# Autodesk Inventor assembly: UltrasonicAssembly
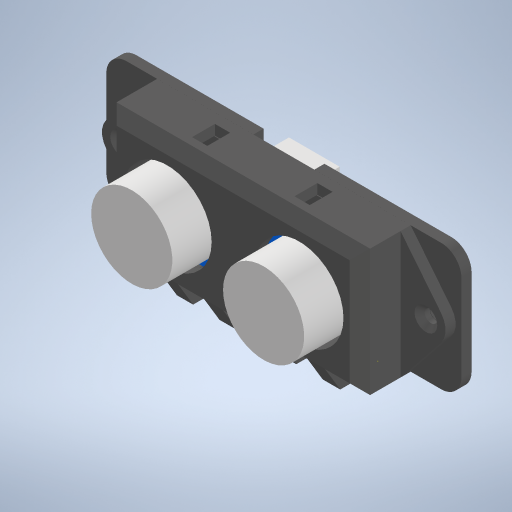
[picture p0: Inventor's stored thumbnail of the model, 512x512]
Saved by Autodesk Inventor 2024.2 (Build 282272000, 272)
## iProperties
Created: 2024-05-04
Part Number: UltrasonicAssembly
Document SubType Name: Assembly
Designer: ringl
Author: ringl
## Documents named in this file (4)
- C:\Users\ringl\OneDrive\Uni_PC_backup\Y4S2\EE579\Assignment\EE579-Skittles\CAD\Assembly\Main\UltrasonicAssembly.iam
- C:\Users\ringl\OneDrive\Uni_PC_backup\Y4S2\EE579\Assignment\EE579-Skittles\CAD\UltrasonicSensorMount02.ipt
- C:\Users\ringl\OneDrive\Uni_PC_backup\Y4S2\EE579\Assignment\EE579-Skittles\CAD\Components\UltrasonicSensor.ipt
- C:\Users\ringl\OneDrive\Uni_PC_backup\Y4S2\EE579\Assignment\EE579-Skittles\CAD\UltrasonicSensorMount_backplate03.ipt
## Components (3 placed, 3 different names)
1. UltrasonicSensorMount02:1 — Mate:3, Mate:4, Mate:5, Mate:6, Mate:7, Mate:8
2. UltrasonicSensorMount_backplate03:1 — Mate:3, Mate:4, Mate:5
3. UltrasonicSensor:1 — Mate:6, Mate:7, Mate:8
## Relationships (6: Mate 6)
- Mate:3: UltrasonicSensorMount02:1 ↔ UltrasonicSensorMount_backplate03:1
- Mate:4: UltrasonicSensorMount02:1 ↔ UltrasonicSensorMount_backplate03:1
- Mate:5: UltrasonicSensorMount02:1 ↔ UltrasonicSensorMount_backplate03:1
- Mate:6: UltrasonicSensorMount02:1 ↔ UltrasonicSensor:1
- Mate:7: UltrasonicSensorMount02:1 ↔ UltrasonicSensor:1
- Mate:8: UltrasonicSensorMount02:1 ↔ UltrasonicSensor:1
